# Autodesk Inventor assembly: Inverter Axle Combineinator
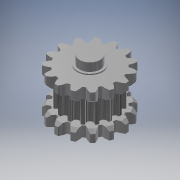
[picture p0: Inventor's stored thumbnail of the model, 180x180]
Saved by Autodesk Inventor 2019.4 (Build 234330000, 330)
## iProperties
Created: 2020-02-16
Part Number: Inverter Axle Combineinator
Document SubType Name: Assembly
Designer: admin
Author: admin
## Documents named in this file (3)
- C:\Users\admin\Desktop\FRC 2020 Engineering\GitHub\7738-2020\Robot V2\Storage System\3D printed Alternator\Inverter Axle Combineinator.iam
- C:\Users\admin\Desktop\FRC 2020 Engineering\GitHub\7738-2020\Robot V2\Storage System\3D printed Alternator\Inverter Axle Combineinator\Design Accelerator\Spur Gears1.iam
- C:\Users\admin\Desktop\FRC 2020 Engineering\GitHub\7738-2020\Robot V2\Storage System\3D printed Alternator\Axle Pulley.ipt
## Components (3 placed, 2 different names)
1. Spur Gears:1 [sub-assembly] — Mate:6, Mate:7, Mate:8, Mate:10
2. Spur Gears:2 [sub-assembly] — Mate:6, Mate:9, Mate:10
3. Axle Pulley:1 — Mate:7, Mate:8, Mate:9
## Relationships (5: Mate 5)
- Mate:6: Spur Gears:1 ↔ Spur Gears:2
- Mate:7: Spur Gears:1 ↔ Axle Pulley:1
- Mate:8: Spur Gears:1 ↔ Axle Pulley:1
- Mate:9: Spur Gears:2 ↔ Axle Pulley:1
- Mate:10: Spur Gears:1 ↔ Spur Gears:2
